# Autodesk Inventor assembly: A_3Way-40
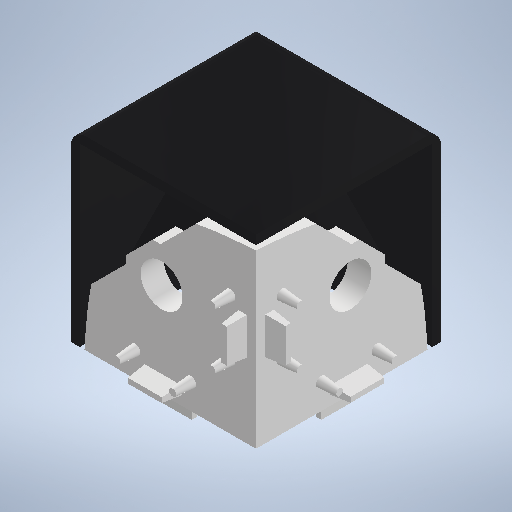
[picture p0: Inventor's stored thumbnail of the model, 512x512]
Saved by Autodesk Inventor 2025.3 (Build 293356000, 356)
## iProperties
Created: 2026-07-28
Part Number: A_3Way-40
Document SubType Name: Assembly
Designer: louis
Author: louis
## Documents named in this file (3)
- C:\Users\louis\OneDrive\Desktop\R_Trident\02_CAD\01_Standard_Parts\03_FRM_Fastener\A_3Way-40.iam
- C:\Users\louis\OneDrive\Desktop\R_Trident\02_CAD\01_Standard_Parts\03_FRM_Fastener\3Way-40.ipt
- C:\Users\louis\OneDrive\Desktop\R_Trident\02_CAD\01_Standard_Parts\03_FRM_Fastener\3Way-40_cover.ipt
## Components (2 placed, 2 different names)
1. 3Way-40:1 — Flush:1, Flush:2, Flush:3
2. 3Way-40_cover:1 — Flush:1, Flush:2, Flush:3
## Relationships (3: Flush 3)
- Flush:1: 3Way-40:1 ↔ 3Way-40_cover:1
- Flush:2: 3Way-40:1 ↔ 3Way-40_cover:1
- Flush:3: 3Way-40:1 ↔ 3Way-40_cover:1
